# Autodesk Inventor assembly: Blue Alliance Arm
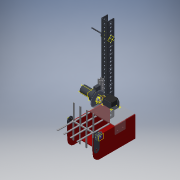
[picture p0: Inventor's stored thumbnail of the model, 180x180]
Saved by Autodesk Inventor 2016 (Build 200138000, 138)
## iProperties
Created: 2015-12-20
Part Number: Blue Alliance Arm
Document SubType Name: Assembly
Designer: tbloo
Author: tbloo
## Documents named in this file (12)
- C:\Users\tbloo\Documents\GitHub\phi_robotics\3d-models\FTC_Tetrix_KOP_Block_Party\Tim Bloot Designs\JAr JaR Bot\Red Alliance Arm.iam
- C:\Users\tbloo\Documents\GitHub\phi_robotics\3d-models\FTC_Tetrix_KOP_Block_Party\Tim Bloot Designs\JAr JaR Bot\Blue Alliance Bucket.iam
- C:\Users\tbloo\Documents\GitHub\phi_robotics\3d-models\FTC_Tetrix_KOP_Block_Party\Tetrix_Kit_FTC\Autodesk Inventor Files\tetrix_axle.ipt
- C:\Users\tbloo\Documents\GitHub\phi_robotics\3d-models\FTC_Tetrix_KOP_Block_Party\Tetrix_Kit_FTC\Autodesk Inventor Files\tetrix_c_channel-5.ipt
- C:\Users\tbloo\Documents\GitHub\phi_robotics\3d-models\FTC_Tetrix_KOP_Block_Party\Tetrix_Kit_FTC\Autodesk Inventor Files\tetrix_axle_lock.iam
- C:\Users\tbloo\Documents\GitHub\phi_robotics\3d-models\FTC_Tetrix_KOP_Block_Party\Tetrix_Kit_FTC\Autodesk Inventor Files\tetrix_c_channel-1.ipt
- C:\Users\tbloo\Documents\GitHub\phi_robotics\3d-models\FTC_Tetrix_KOP_Block_Party\Tim Bloot Designs\JAr JaR Bot\cube channel short.ipt
- C:\Users\tbloo\Documents\GitHub\phi_robotics\3d-models\FTC_Tetrix_KOP_Block_Party\Tetrix_Kit_FTC\Autodesk Inventor Files\tetrix_motor_mount-old.ipt
- C:\Users\tbloo\Documents\GitHub\phi_robotics\3d-models\FTC_Tetrix_KOP_Block_Party\Tetrix_Kit_FTC\Autodesk Inventor Files\tetrix_motor.iam
- C:\Users\tbloo\Documents\GitHub\phi_robotics\3d-models\FTC_Tetrix_KOP_Block_Party\Tetrix_Kit_FTC\Autodesk Inventor Files\tetrix_maxle_lock.iam
- C:\Users\tbloo\Documents\GitHub\phi_robotics\3d-models\FTC_Tetrix_KOP_Block_Party\Tetrix_Kit_FTC\Autodesk Inventor Files\tetrix_chain_gear-32t.ipt
- C:\Users\tbloo\Documents\GitHub\phi_robotics\3d-models\FTC_Tetrix_KOP_Block_Party\Tetrix_Kit_FTC\Autodesk Inventor Files\tetrix_screw.ipt
## Components (14 placed, 11 different names)
1. Blue Alliance Bucket:1 [sub-assembly] — Mate:1, Flush:1, Flush:2
2. tetrix_axle:1 — Rigid:1
3. tetrix_c_channel-5:1 — Rigid:2, Rigid:3, Rigid:4, Rigid:5, Rigid:6
4. tetrix_axle_lock:1 [sub-assembly] — Rigid:3
5. tetrix_axle_lock:2 [sub-assembly] — Rigid:1, Rigid:2
6. tetrix_c_channel-1:1 — Rigid:4
7. tetrix_c_channel-1:2 — Rigid:5, Mate:1, Flush:1, Flush:2
8. cube channel short:1 — Rigid:6, Rigid:12
9. tetrix_motor_mount-old:1 — Rigid:12, Rotational:1
10. tetrix_motor:1 [sub-assembly] — Rigid:11, Rotational:1
11. tetrix_maxle_lock:1 [sub-assembly] — Rigid:8, Rigid:11
12. tetrix_chain_gear-32t:1 — Rigid:8, Rigid:9, Rigid:10
13. tetrix_screw:1 — Rigid:10
14. tetrix_screw:2 — Rigid:9
## Relationships (15: WeldJoint 11, Flush 2, Mate 1, RevoluteJoint 1)
- Rigid:1 [WeldJoint]: tetrix_axle:1 ↔ tetrix_axle_lock:2
- Rigid:2 [WeldJoint]: tetrix_c_channel-5:1 ↔ tetrix_axle_lock:2
- Rigid:3 [WeldJoint]: tetrix_c_channel-5:1 ↔ tetrix_axle_lock:1
- Rigid:4 [WeldJoint]: tetrix_c_channel-5:1 ↔ tetrix_c_channel-1:1
- Rigid:5 [WeldJoint]: tetrix_c_channel-5:1 ↔ tetrix_c_channel-1:2
- Mate:1: Blue Alliance Bucket:1 ↔ tetrix_c_channel-1:2
- Flush:1: Blue Alliance Bucket:1 ↔ tetrix_c_channel-1:2
- Flush:2: Blue Alliance Bucket:1 ↔ tetrix_c_channel-1:2
- Rigid:6 [WeldJoint]: tetrix_c_channel-5:1 ↔ cube channel short:1
- Rigid:8 [WeldJoint]: tetrix_maxle_lock:1 ↔ tetrix_chain_gear-32t:1
- Rigid:9 [WeldJoint]: tetrix_chain_gear-32t:1 ↔ tetrix_screw:2
- Rigid:10 [WeldJoint]: tetrix_chain_gear-32t:1 ↔ tetrix_screw:1
- Rigid:11 [WeldJoint] (-7 mm): tetrix_motor:1 ↔ tetrix_maxle_lock:1
- Rigid:12 [WeldJoint]: cube channel short:1 ↔ tetrix_motor_mount-old:1
- Rotational:1 [RevoluteJoint]: tetrix_motor_mount-old:1 ↔ tetrix_motor:1
